# Autodesk Inventor assembly: extension arm spool 2_75
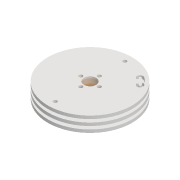
[picture p0: Inventor's stored thumbnail of the model, 180x180]
Saved by Autodesk Inventor 2020 (Build 240168000, 168)
## iProperties
Created: 2020-01-04
Part Number: extension arm spool 2_75
Document SubType Name: Assembly
Designer: ball
Author: ball
## Documents named in this file (3)
- C:\FTC\FTC8863CAD\2019 Robot\Delivery\extension arm\extension arm spool 2_75.iam
- C:\FTC\FTC8863CAD\2019 Robot\Delivery\extension arm\3_5 in spool outer plate.ipt
- C:\FTC\FTC8863CAD\2019 Robot\Delivery\extension arm\2_75 in spool inner plate.ipt
## Components (5 placed, 2 different names)
1. 3_5 in spool outer plate:1 — Mate:1, Mate:2, Mate:3
2. 3_5 in spool outer plate:2 — Mate:4, Mate:5, Mate:6, Mate:7, Mate:8, Mate:9
3. 2_75 in spool inner plate:1 — Mate:1, Mate:2, Mate:3, Mate:4, Mate:5, Mate:6
4. 2_75 in spool inner plate:2 — Mate:7, Mate:8, Mate:9, Mate:10, Mate:11, Mate:12
5. 3_5 in spool outer plate:3 — Mate:10, Mate:11, Mate:12
## Relationships (12: Mate 12)
- Mate:1: 3_5 in spool outer plate:1 ↔ 2_75 in spool inner plate:1
- Mate:2: 3_5 in spool outer plate:1 ↔ 2_75 in spool inner plate:1
- Mate:3: 3_5 in spool outer plate:1 ↔ 2_75 in spool inner plate:1
- Mate:4: 3_5 in spool outer plate:2 ↔ 2_75 in spool inner plate:1
- Mate:5: 3_5 in spool outer plate:2 ↔ 2_75 in spool inner plate:1
- Mate:6: 3_5 in spool outer plate:2 ↔ 2_75 in spool inner plate:1
- Mate:7: 3_5 in spool outer plate:2 ↔ 2_75 in spool inner plate:2
- Mate:8: 3_5 in spool outer plate:2 ↔ 2_75 in spool inner plate:2
- Mate:9: 3_5 in spool outer plate:2 ↔ 2_75 in spool inner plate:2
- Mate:10: 2_75 in spool inner plate:2 ↔ 3_5 in spool outer plate:3
- Mate:11: 2_75 in spool inner plate:2 ↔ 3_5 in spool outer plate:3
- Mate:12: 2_75 in spool inner plate:2 ↔ 3_5 in spool outer plate:3
